# Autodesk Inventor assembly: PCB_R2D2
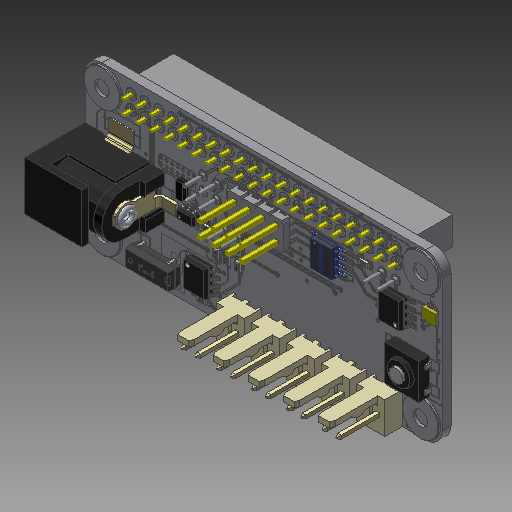
[picture p0: Inventor's stored thumbnail of the model, 512x512]
Saved by Autodesk Inventor 2017 (Build 210142000, 142)
## iProperties
Created: 2017-10-14
Part Number: PCB_R2D2
Description: PCB Design
Document SubType Name: Assembly
Designer: P. Baesso
Sending System: allegro_16.6-2015S079
Preprocessor: ST-DEVELOPER v15
Title: R2D2
Author: phpgb
## Documents named in this file (5)
- C:\Rymapt\ethoscope_hardware\Shield\Files\PCB_R2D2.iam
- C:\Rymapt\ethoscope_hardware\Shield\Files\PCB_BOARD.ipt
- C:\Rymapt\ethoscope_hardware\Shield\Files\PCB_EXTERNAL COPPER.iam
- C:\Rymapt\ethoscope_hardware\Shield\Files\PCB_COMPONENTS.iam
- C:\Rymapt\ethoscope_hardware\Shield\Files\BCS-120-F-D-TE.ipt
## Components (4 placed, 4 different names)
1. BOARD — Mate:1, Mate:2, Mate:3, Angle:1
2. EXTERNAL COPPER [sub-assembly]
3. COMPONENTS [sub-assembly]
4. BCS-120-F-D-TE:1 — Mate:1, Mate:2, Mate:3, Angle:1
## Relationships (4: Mate 3, Angle 1)
- Mate:1: BOARD ↔ BCS-120-F-D-TE:1
- Mate:2 (-0.125 mm): BOARD ↔ BCS-120-F-D-TE:1
- Mate:3 (-0.245 mm): BOARD ↔ BCS-120-F-D-TE:1
- Angle:1 (0 deg): BOARD ↔ BCS-120-F-D-TE:1
